# Autodesk Inventor assembly: Lift
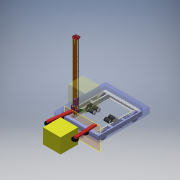
[picture p0: Inventor's stored thumbnail of the model, 180x180]
Saved by Autodesk Inventor 2017 SP1 (Build 210196100, 196)
## iProperties
Created: 2018-01-18
Part Number: Lift
Document SubType Name: Assembly
Designer: Ben
Mass: 3205.42 g
Surface Area: 51290.7 cm^2
Volume: 100604 cm^3
Density: 0.0318616 g/cm^3
Author: Ben
## Documents named in this file (19)
- C:\Users\Ben\Desktop\Projects\2018 Robot\Cube Lift\Lift.iam
- C:\Users\Ben\Desktop\Projects\2018 Robot\Cube Lift\Rail.ipt
- C:\Users\Ben\Desktop\Projects\2018 Robot\Chassis\2018_chassis.iam
- C:\Users\Ben\Desktop\Projects\2018 Robot\Cube Lift\roller bushing.iam
- C:\Users\Ben\Desktop\Projects\2018 Robot\Cube Lift\cube.ipt
- C:\Users\Ben\Desktop\Projects\2018 Robot\Cube Lift\carriage plate square 2.ipt
- C:\Users\Ben\Desktop\Projects\2018 Robot\Cube Lift\support plate.ipt
- C:\Users\Ben\Desktop\Projects\2018 Robot\Cube Lift\support L.ipt
- C:\Users\Ben\Desktop\Projects\2018 Robot\Cube Lift\top pully bracket.ipt
- C:\Users\Ben\Desktop\Projects\2018 Robot\Cube Lift\pulley XL 1in.ipt
- C:\Users\Ben\Desktop\Projects\2018 Robot\Cube Lift\pulley XL 1.375in 2.ipt
- C:\Users\Ben\Desktop\Projects\2018 Robot\Cube Lift\first stage belt.ipt
- C:\Users\Ben\Desktop\Projects\2018 Robot\Cube Lift\roller plate.ipt
- C:\Users\Ben\Desktop\Projects\2018 Robot\Cube Lift\pulley XL 1.25in.ipt
- C:\Users\Ben\Desktop\Projects\2018 Robot\Cube Lift\upper anchor.ipt
- C:\Users\Ben\Desktop\Projects\2018 Robot\Cube Lift\top pully bracket 2.ipt
- C:\Users\Ben\Desktop\Projects\2018 Robot\Cube Lift\second stage belt 2.ipt
- C:\Users\Ben\Desktop\Projects\2018 Robot\Cube Lift\carriage plate for intake.ipt
- C:\Users\Ben\Desktop\Projects\2018 Robot\Cube Intake\Intake.iam
## Components (28 placed, 18 different names)
1. Rail:1 — Mate:13, Flush:15, Flush:16, Mate:20, Mate:21, Mate:22, Mate:23, Mate:30, Mate:32, Flush:25, Mate:33, Flush:26, Flush:27, Flush:28, Flush:29, Mate:39, Flush:30, Angle:2, Flush:33, Mate:44
2. 2018_chassis:1 [sub-assembly] — Mate:1, Flush:3, Flush:4, Mate:13, Flush:15, Flush:21, Insert:7, Angle:1, Mate:31
3. Rail:3 — Mate:5, Flush:16, Mate:24, Mate:41, Angle:3, Flush:32, Mate:45, Flush:34, Mate:48, Flush:35, Angle:4, Mate:50
4. roller bushing:1 [sub-assembly] — Mate:38, Flush:28
5. cube:1 — Flush:5
6. cube:2 — Flush:6, Mate:26
7. carriage plate square 2:1 — Mate:5, Mate:20, Mate:21, Mate:22, Mate:23, Mate:24, Mate:34, Mate:35, Mate:36, Mate:37, Mate:38, Mate:42, Mate:43
8. roller bushing:2 [sub-assembly] — Mate:36, Flush:26
9. roller bushing:3 [sub-assembly] — Mate:37, Flush:27
10. roller bushing:4 [sub-assembly]
11. roller bushing:5 [sub-assembly]
12. roller bushing:6 [sub-assembly]
13. support plate:1 — Insert:7, Angle:1, Mate:30, Insert:8
14. support L:1 — Mate:31, Mate:32, Flush:25
15. carriage plate square 2:3 — Mate:33, Mate:34, Mate:35
16. top pully bracket:1 — Flush:29, Mate:39, Flush:30, Mate:40, Flush:31
17. pulley XL 1in:1 — Insert:8, Insert:9
18. pulley XL 1.375in 2:1 — Mate:40, Flush:31
19. first stage belt:1 — Insert:9, Angle:2
20. roller plate:1 — Mate:41, Angle:3, Mate:42
21. pulley XL 1.25in:1 — Flush:32, Mate:43, Insert:10
22. upper anchor:1 — Flush:33, Mate:44
23. carriage plate square 2:4 — Mate:45, Mate:51, Mate:52
24. top pully bracket 2:1 — Flush:34, Mate:48, Flush:35, Mate:49, Flush:36
25. pulley XL 1.25in:2 — Mate:49, Flush:36
26. second stage belt 2:1 — Insert:10, Angle:4
27. carriage plate for intake:1 — Mate:50, Mate:51, Mate:52
28. Intake:1 [sub-assembly] — Flush:37, Flush:38
## Relationships (62: Mate 30, Flush 24, Insert 4, Angle 4)
- Mate:1 (44.45 mm): 2018_chassis:1
- Flush:3: 2018_chassis:1
- Flush:4: 2018_chassis:1
- Flush:5: cube:1
- Flush:6: cube:2
- Mate:5: Rail:3 ↔ carriage plate square 2:1
- Mate:13: Rail:1 ↔ 2018_chassis:1
- Flush:15 (127 mm): Rail:1 ↔ 2018_chassis:1
- Flush:16: Rail:1 ↔ Rail:3
- Mate:20 (9.525 mm): Rail:1 ↔ carriage plate square 2:1
- Mate:21 (13.9192 mm): Rail:1 ↔ carriage plate square 2:1
- Mate:22 (13.9192 mm): Rail:1 ↔ carriage plate square 2:1
- Mate:23 (13.9192 mm): Rail:1 ↔ carriage plate square 2:1
- Mate:24: Rail:3 ↔ carriage plate square 2:1
- Flush:18 (1397 mm)
- Flush:19 (1930.4 mm)
- Flush:20 (2184.4 mm)
- Flush:21 (-609.6 mm): 2018_chassis:1
- Mate:26: cube:2
- Insert:7: 2018_chassis:1 ↔ support plate:1
- Angle:1 (0 deg): 2018_chassis:1 ↔ support plate:1
- Mate:30: Rail:1 ↔ support plate:1
- Mate:31: 2018_chassis:1 ↔ support L:1
- Mate:32: Rail:1 ↔ support L:1
- Flush:25: Rail:1 ↔ support L:1
- Mate:33 (2.3622 mm): Rail:1 ↔ carriage plate square 2:3
- Mate:34: carriage plate square 2:1 ↔ carriage plate square 2:3
- Mate:35: carriage plate square 2:1 ↔ carriage plate square 2:3
- Mate:36: carriage plate square 2:1 ↔ roller bushing:2
- Flush:26 (-2.3622 mm): Rail:1 ↔ roller bushing:2
- Mate:37: carriage plate square 2:1 ↔ roller bushing:3
- Flush:27 (-2.3622 mm): Rail:1 ↔ roller bushing:3
- Mate:38: roller bushing:1 ↔ carriage plate square 2:1
- Flush:28 (2.3622 mm): Rail:1 ↔ roller bushing:1
- Flush:29 (-1.5875 mm): Rail:1 ↔ top pully bracket:1
- Mate:39: Rail:1 ↔ top pully bracket:1
- Flush:30 (6.35 mm): Rail:1 ↔ top pully bracket:1
- Insert:8 (4.7625 mm): support plate:1 ↔ pulley XL 1in:1
- Mate:40: top pully bracket:1 ↔ pulley XL 1.375in 2:1
- Flush:31: top pully bracket:1 ↔ pulley XL 1.375in 2:1
- Insert:9 (1.5875 mm): pulley XL 1in:1 ↔ first stage belt:1
- Angle:2 (0 deg): Rail:1 ↔ first stage belt:1
- Mate:41: Rail:3 ↔ roller plate:1
- Angle:3 (0 deg): Rail:3 ↔ roller plate:1
- Flush:32: Rail:3 ↔ pulley XL 1.25in:1
- Mate:42: carriage plate square 2:1 ↔ roller plate:1
- Mate:43: carriage plate square 2:1 ↔ pulley XL 1.25in:1
- Flush:33: Rail:1 ↔ upper anchor:1
- Mate:44: Rail:1 ↔ upper anchor:1
- Mate:45 (2.3622 mm): Rail:3 ↔ carriage plate square 2:4
- Flush:34 (-1.5875 mm): Rail:3 ↔ top pully bracket 2:1
- Mate:48: Rail:3 ↔ top pully bracket 2:1
- Flush:35 (-6.35 mm): Rail:3 ↔ top pully bracket 2:1
- Mate:49: top pully bracket 2:1 ↔ pulley XL 1.25in:2
- Flush:36: top pully bracket 2:1 ↔ pulley XL 1.25in:2
- Insert:10 (3.175 mm): pulley XL 1.25in:1 ↔ second stage belt 2:1
- Angle:4 (0 deg): Rail:3 ↔ second stage belt 2:1
- Mate:50 (2.3622 mm): Rail:3 ↔ carriage plate for intake:1
- Mate:51: carriage plate square 2:4 ↔ carriage plate for intake:1
- Mate:52: carriage plate square 2:4 ↔ carriage plate for intake:1
- Flush:37: Intake:1
- Flush:38: Intake:1
